# Autodesk Inventor assembly: ASY DMF filter package v2.1
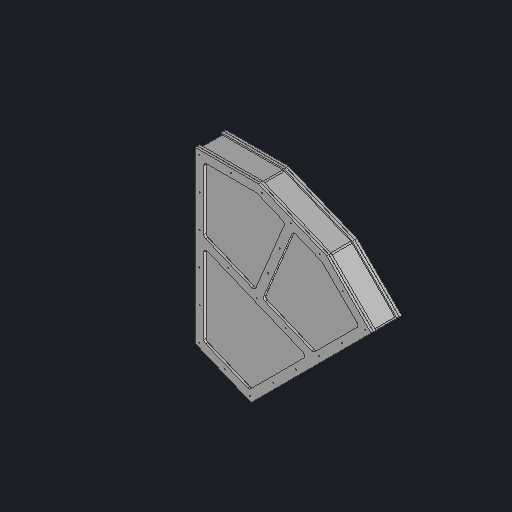
[picture p0: Inventor's stored thumbnail of the model, 512x512]
Saved by Autodesk Inventor 2026.2 (Build 302298000, 298)
## iProperties
Created: 2024-05-16
Part Number: ASY DMF filter package v2.1
Document SubType Name: Assembly
Designer: admin
Author: admin
## Documents named in this file (13)
- C:\Users\admin\Documents\Inventor\DMF-Disk-Micro-Filter\Барабан v2.1\ASY DMF filter package v2.1.iam
- C:\Users\admin\Documents\Inventor\DMF-Disk-Micro-Filter\Барабан v2.1\DMF 01 51 outside frame v2.1.ipt
- ДМС 201 Внешняя рамка.ipt
- C:\Users\admin\Documents\Inventor\DMF-Disk-Micro-Filter\Барабан v2.1\DMF 01 52 Top sheet v2.1.ipt
- C:\Users\admin\Documents\Inventor\DMF-Disk-Micro-Filter\Барабан v2.1\DMF 01 53 side part v2.1.ipt
- C:\Users\admin\Documents\Inventor\DMF-Disk-Micro-Filter\Барабан v2.1\DMF 01 54 lower sheet v2.1.ipt
- C:\Users\admin\Documents\Inventor\DMF-Disk-Micro-Filter\Барабан v2.1\DMF 01 56 Крепление сетки к кассете v2.1.ipt
- ДМС 206 Крепление сетки к кассете.ipt
- C:\Users\admin\Documents\Inventor\DMF-Disk-Micro-Filter\Барабан v2.1\DMF 01 57 Сетка кассеты v2.1.ipt
- ДМС 207 Сетка кассеты.ipt
- C:\Users\admin\Documents\Inventor\DMF-Disk-Micro-Filter\Барабан v2.1\DMF 01 51 outside frame_MIR1 v2.1.ipt
- C:\Users\admin\Documents\Inventor\DMF-Disk-Micro-Filter\Барабан v2.1\DMF 01 56 Крепление сетки к кассете_MIR1 v2.1.ipt
- C:\Users\admin\Documents\Inventor\DMF-Disk-Micro-Filter\Барабан v2.1\DMF 01 57 Сетка кассеты_MIR1 v2.1.ipt
## Components (10 placed, 9 different names)
1. DMF 01 51 outside frame v2.1.ipt:1
2. DMF 01 52 Top sheet v2.1.ipt:1 — Rigid:7
3. DMF 01 53 side part v2.1.ipt:1
4. DMF 01 54 lower sheet v2.1.ipt:1
5. DMF 01 56 Крепление сетки к кассете v2.1.ipt:1
6. DMF 01 57 Сетка кассеты v2.1.ipt:1
7. DMF 01 53 side part v2.1.ipt:2
8. DMF 01 51 outside frame_MIR1 v2.1.ipt:1 — Rigid:7
9. DMF 01 56 Крепление сетки к кассете_MIR1 v2.1.ipt:1
10. DMF 01 57 Сетка кассеты_MIR1 v2.1.ipt:1
## Relationships (13: WeldJoint 7, Mate 3, RevoluteJoint 2, Flush 1)
- [Mate]: DMF 01 51 outside frame v2.1.ipt:1
- [Flush]: DMF 01 56 Крепление сетки к кассете v2.1.ipt:1
- [WeldJoint]: DMF 01 51 outside frame v2.1.ipt:1 ↔ DMF 01 57 Сетка кассеты v2.1.ipt:1
- [WeldJoint]: DMF 01 51 outside frame v2.1.ipt:1 ↔ DMF 01 52 Top sheet v2.1.ipt:1
- [RevoluteJoint]: DMF 01 51 outside frame v2.1.ipt:1 ↔ DMF 01 53 side part v2.1.ipt:1
- [Mate]: DMF 01 51 outside frame v2.1.ipt:1 ↔ DMF 01 53 side part v2.1.ipt:1
- [WeldJoint] (0.5 mm): DMF 01 51 outside frame v2.1.ipt:1 ↔ DMF 01 56 Крепление сетки к кассете v2.1.ipt:1
- [RevoluteJoint]: DMF 01 51 outside frame v2.1.ipt:1 ↔ DMF 01 53 side part v2.1.ipt:2
- [Mate]: DMF 01 51 outside frame v2.1.ipt:1 ↔ DMF 01 53 side part v2.1.ipt:2
- [WeldJoint]: DMF 01 51 outside frame v2.1.ipt:1 ↔ DMF 01 54 lower sheet v2.1.ipt:1
- [WeldJoint] (0.5 mm): DMF 01 51 outside frame_MIR1 v2.1.ipt:1 ↔ DMF 01 56 Крепление сетки к кассете_MIR1 v2.1.ipt:1
- [WeldJoint]: DMF 01 51 outside frame_MIR1 v2.1.ipt:1 ↔ DMF 01 57 Сетка кассеты_MIR1 v2.1.ipt:1
- Rigid:7 [WeldJoint]: DMF 01 52 Top sheet v2.1.ipt:1 ↔ DMF 01 51 outside frame_MIR1 v2.1.ipt:1
## Named parameters: d0_d1 = 0 mm, d1_d3 = 0 mm, d2_d4 = 0 mm, d3_d5 = 90 deg, d4_d6 = 0 mm, d5_d7 = 0.5 mm, d6_d8 = 0 mm, d7_d9 = -90 deg, d8_d10 = 0 mm, d9_d11 = 0 mm
